# Autodesk Inventor assembly: EnsembleV1
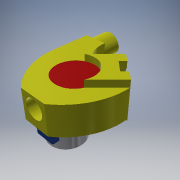
[picture p0: Inventor's stored thumbnail of the model, 180x180]
Saved by Autodesk Inventor 2019 (Build 230136000, 136)
## iProperties
Created: 2020-12-14
Part Number: EnsembleV1
Material: Générique
Document SubType Name: Assembly
Designer: tom.mousset
Author: tom.mousset
## Documents named in this file (4)
- F:\triSmarties\EnsembleV1.iam
- F:\triSmarties\carcasseHaut.ipt
- F:\triSmarties\roue.ipt
- F:\triSmarties\Step - 28BYJ-48.ipt
## Components (3 placed, 3 different names)
1. carcasseHaut:1 — Placage:1, Placage:2, Placage:4, Placage:5, Angle:2
2. Step - 28BYJ-48:1 — Placage:1, Placage:2, Angle:1, Angle:2
3. roue:1 — Placage:4, Placage:5, Angle:1
## Relationships (6: Mate 4, Angle 2)
- Placage:1 [Mate]: carcasseHaut:1 ↔ Step - 28BYJ-48:1
- Placage:2 [Mate]: carcasseHaut:1 ↔ Step - 28BYJ-48:1
- Placage:4 [Mate]: carcasseHaut:1 ↔ roue:1
- Placage:5 [Mate]: carcasseHaut:1 ↔ roue:1
- Angle:1 (45 deg): Step - 28BYJ-48:1 ↔ roue:1
- Angle:2 (180 deg): carcasseHaut:1 ↔ Step - 28BYJ-48:1
